# Autodesk Inventor assembly: am-940a-6-HiGrip-
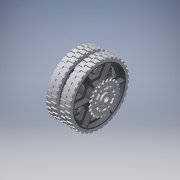
[picture p0: Inventor's stored thumbnail of the model, 180x180]
Saved by Autodesk Inventor 2016 (Build 200138000, 138)
## iProperties
Created: 2014-03-19
Part Number: am-940a-6-HiGrip-
Description: STEP AP214
Document SubType Name: Assembly
Designer: gus
Mass: 273.861 g
Surface Area: 1275.64 cm^2
Volume: 206.584 cm^3
Density: 1.32567 g/cm^3
Sending System: SolidWorks 2010
Preprocessor: SwSTEP 2.0
Title: 6-HiGrip-am-940aSTEP.STEP
Revision Number: ANY
## Documents named in this file (6)
- \\Mac\Home\Desktop\2016 robot cad\chassis\am-940a-6-HiGrip-.iam
- \\Mac\Home\Desktop\2016 robot cad\chassis\6 wheel Rev 4.ipt
- \\Mac\Home\Desktop\2016 robot cad\chassis\6 wheel tread II.ipt
- \\Mac\Home\Desktop\2016 robot cad\chassis\am-0077a-500 Key Hub r2.ipt
- \\Mac\Home\Desktop\2016 robot cad\chassis\24tsprocket.ipt
- \\Mac\Home\Desktop\2016 robot cad\chassis\shaftcollar.ipt
## Components (7 placed, 7 different names)
1. 6 wheel Rev 4_1 — Mate:1, Flush:1, Cylindrical:1, Mate:2, Mate:6, Mate:7, Mate:8
2. 6 wheel tread II_2 — Mate:1, Flush:1
3. am-0077a-500 Key Hub r2:1 — Cylindrical:1, Mate:2, Cylindrical:2, Mate:3, Mate:4, Rotational:1
4. 24tsprocket:1 — Cylindrical:2, Mate:3, Mate:4
5. shaftcollar:1 — Rotational:1
6. 6 wheel tread II:2 — Mate:5, Flush:2
7. 6 wheel Rev 4:2 — Mate:5, Flush:2, Mate:6, Mate:7, Mate:8
## Relationships (13: Mate 8, Flush 2, CylindricalJoint 2, RevoluteJoint 1)
- Mate:1: 6 wheel Rev 4_1 ↔ 6 wheel tread II_2
- Flush:1: 6 wheel Rev 4_1 ↔ 6 wheel tread II_2
- Cylindrical:1: 6 wheel Rev 4_1 ↔ am-0077a-500 Key Hub r2:1
- Mate:2: 6 wheel Rev 4_1 ↔ am-0077a-500 Key Hub r2:1
- Cylindrical:2: am-0077a-500 Key Hub r2:1 ↔ 24tsprocket:1
- Mate:3: am-0077a-500 Key Hub r2:1 ↔ 24tsprocket:1
- Mate:4: am-0077a-500 Key Hub r2:1 ↔ 24tsprocket:1
- Rotational:1 [RevoluteJoint]: am-0077a-500 Key Hub r2:1 ↔ shaftcollar:1
- Mate:5: 6 wheel tread II:2 ↔ 6 wheel Rev 4:2
- Flush:2: 6 wheel tread II:2 ↔ 6 wheel Rev 4:2
- Mate:6: 6 wheel Rev 4_1 ↔ 6 wheel Rev 4:2
- Mate:7: 6 wheel Rev 4_1 ↔ 6 wheel Rev 4:2
- Mate:8: 6 wheel Rev 4_1 ↔ 6 wheel Rev 4:2
